# Autodesk Inventor assembly: Display
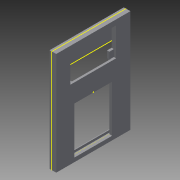
[picture p0: Inventor's stored thumbnail of the model, 180x180]
Saved by Autodesk Inventor 2014 SP1 (Build 180222100, 222)
## iProperties
Created: 2014-03-24
Part Number: Display
Document SubType Name: Assembly
Designer: patrigg
Author: patrigg
## Documents named in this file (3)
- C:\Users\patrigg\Documents\Promotion\Implementierung\3D Display\3D Model\Display.iam
- C:\Users\patrigg\Documents\Promotion\Implementierung\3D Display\3D Model\Case.ipt
- C:\Users\patrigg\Documents\Promotion\Implementierung\3D Display\3D Model\DisplayCase.ipt
## Components (2 placed, 2 different names)
1. DisplayCase:1 — Rigid:1
2. Case:3 — Rigid:1
## Relationships (1: WeldJoint 1)
- Rigid:1 [WeldJoint]: DisplayCase:1 ↔ Case:3
